# Autodesk Inventor assembly: Assembly
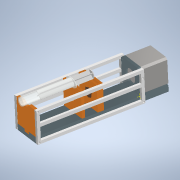
[picture p0: Inventor's stored thumbnail of the model, 180x180]
Saved by Autodesk Inventor 2021.2 (Build 252289000, 289)
## iProperties
Created: 2024-04-20
Part Number: Assembly
Document SubType Name: Assembly
Designer: cioba
Author: cioba
## Documents named in this file (14)
- C:\Users\cioba\OneDrive\Desktop\syringe\Assembly.iam
- C:\Users\cioba\OneDrive\Desktop\syringe\sina.ipt
- C:\Users\cioba\OneDrive\Desktop\syringe\motor.ipt
- C:\Users\cioba\OneDrive\Desktop\syringe\attachment motor.ipt
- C:\Users\cioba\OneDrive\Desktop\syringe\gaica cu suportul.ipt
- C:\Users\cioba\OneDrive\Desktop\syringe\gaica.ipt
- C:\Users\cioba\OneDrive\Desktop\syringe\suport cu rulment pentru tija.ipt
- C:\Users\cioba\OneDrive\Desktop\syringe\suport continuare seringa.ipt
- C:\Users\cioba\OneDrive\Desktop\syringe\seringa outer.ipt
- C:\Users\cioba\OneDrive\Desktop\syringe\seringa inside.ipt
- C:\Users\cioba\OneDrive\Desktop\syringe\motor-tija prindere.ipt
- C:\Users\cioba\OneDrive\Desktop\syringe\tija filet.ipt
- C:\Users\cioba\OneDrive\Desktop\syringe\lateral suport 2.ipt
- C:\Users\cioba\OneDrive\Desktop\syringe\lateral suport.ipt
## Components (13 placed, 13 different names)
1. sina:1 — Mate:1, Flush:1, Mate:4, Mate:5, Mate:6, Mate:9, Mate:10, Mate:11, Mate:14, Mate:18, Mate:19, Mate:20, Mate:21, Mate:24, Mate:25
2. motor:1 — Mate:1, Flush:1, Mate:2, Mate:3, Mate:14, Insert:1
3. attachment motor:1 — Mate:2, Mate:3
4. gaica cu suportul:1 — Mate:4, Mate:5, Mate:6, Mate:7, Mate:8, Mate:22
5. gaica:1 — Mate:7, Mate:8
6. suport cu rulment pentru tija:1 — Mate:9, Mate:10, Mate:11
7. suport continuare seringa:1 — Mate:16, Mate:18, Mate:19, Mate:20, Mate:21, Mate:23, Mate:26
8. seringa outer:1 — Mate:15, Mate:16
9. seringa inside:1 — Mate:15, Mate:22
10. motor-tija prindere:1 — Insert:1, Insert:2
11. tija filet:1 — Insert:2
12. lateral suport 2:1 — Mate:23, Mate:24
13. lateral suport:1 — Mate:25, Mate:26
## Relationships (26: Mate 23, Insert 2, Flush 1)
- Mate:1: sina:1 ↔ motor:1
- Flush:1: sina:1 ↔ motor:1
- Mate:2: motor:1 ↔ attachment motor:1
- Mate:3: motor:1 ↔ attachment motor:1
- Mate:4: sina:1 ↔ gaica cu suportul:1
- Mate:5: sina:1 ↔ gaica cu suportul:1
- Mate:6: sina:1 ↔ gaica cu suportul:1
- Mate:7: gaica cu suportul:1 ↔ gaica:1
- Mate:8: gaica cu suportul:1 ↔ gaica:1
- Mate:9: sina:1 ↔ suport cu rulment pentru tija:1
- Mate:10: sina:1 ↔ suport cu rulment pentru tija:1
- Mate:11: sina:1 ↔ suport cu rulment pentru tija:1
- Mate:14: sina:1 ↔ motor:1
- Mate:15: seringa outer:1 ↔ seringa inside:1
- Mate:16: suport continuare seringa:1 ↔ seringa outer:1
- Insert:1 (-10 mm): motor:1 ↔ motor-tija prindere:1
- Insert:2 (-10 mm): motor-tija prindere:1 ↔ tija filet:1
- Mate:18: sina:1 ↔ suport continuare seringa:1
- Mate:19: sina:1 ↔ suport continuare seringa:1
- Mate:20: sina:1 ↔ suport continuare seringa:1
- Mate:21: sina:1 ↔ suport continuare seringa:1
- Mate:22: gaica cu suportul:1 ↔ seringa inside:1
- Mate:23: suport continuare seringa:1 ↔ lateral suport 2:1
- Mate:24: sina:1 ↔ lateral suport 2:1
- Mate:25: sina:1 ↔ lateral suport:1
- Mate:26: suport continuare seringa:1 ↔ lateral suport:1
